# Autodesk Inventor assembly: SPE1V1 Estructura
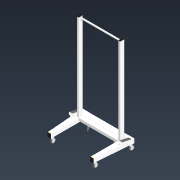
[picture p0: Inventor's stored thumbnail of the model, 180x180]
Saved by Autodesk Inventor 2021.2 (Build 252289000, 289)
## iProperties
Created: 2026-06-02
Part Number: SPE1V1 Estructura
Document SubType Name: Assembly
Designer: nelso
Mass: 32774.5 g
Surface Area: 45303.3 cm^2
Volume: 6303.93 cm^3
Density: 5.19906 g/cm^3
Author: nelso
## Documents named in this file (21)
- C:\Users\Tecnica\OneDrive\Documentos\Mecanica\Soporte-Paciente-Espinografia\Workspace\SPE1V1 Estructura.iam
- C:\Users\Tecnica\OneDrive\Documentos\Mecanica\Soporte-Paciente-Espinografia\Workspace\SP28V1 Tapacanto Delantero.ipt
- C:\Users\Tecnica\OneDrive\Documentos\Mecanica\Soporte-Paciente-Espinografia\Workspace\SP27V1 Tapacanto Superior.ipt
- C:\Users\Tecnica\OneDrive\Documentos\Mecanica\Soporte-Paciente-Espinografia\Workspace\RFPLUS8PO300.ipt
- C:\Users\Tecnica\OneDrive\Documentos\Mecanica\Soporte-Paciente-Espinografia\Workspace\SP26V1 Varilla Pedal.ipt
- C:\Users\Tecnica\OneDrive\Documentos\Mecanica\Soporte-Paciente-Espinografia\Workspace\SP23V1 Pedal Izquierdo.ipt
- C:\Users\Tecnica\OneDrive\Documentos\Mecanica\Soporte-Paciente-Espinografia\Workspace\SPE9V1 Freno.iam
- C:\Users\Tecnica\OneDrive\Documentos\Mecanica\Soporte-Paciente-Espinografia\Workspace\SP22V1 Pedal Derecho.ipt
- C:\Users\Tecnica\OneDrive\Documentos\Mecanica\Soporte-Paciente-Espinografia\Workspace\G3-100-PPP-RU.ipt
- C:\Users\Tecnica\OneDrive\Documentos\Mecanica\Soporte-Paciente-Espinografia\Workspace\DIN 555A10C.ipt
- C:\Users\Tecnica\OneDrive\Documentos\Mecanica\Soporte-Paciente-Espinografia\Workspace\DIN125-A8,4C.ipt
- C:\Users\Tecnica\OneDrive\Documentos\Mecanica\Soporte-Paciente-Espinografia\Workspace\DIN933M8X1.25L20C.ipt
- C:\Users\Tecnica\OneDrive\Documentos\Mecanica\Soporte-Paciente-Espinografia\Workspace\SP25V1 Seguro Pedales.ipt
- C:\Users\Tecnica\OneDrive\Documentos\Mecanica\Soporte-Paciente-Espinografia\Workspace\ISO7380M6X1L12I.ipt
- C:\Users\Tecnica\OneDrive\Documentos\Mecanica\Soporte-Paciente-Espinografia\Workspace\DIN137-B6.ipt
- C:\Users\Tecnica\OneDrive\Documentos\Mecanica\Soporte-Paciente-Espinografia\Workspace\ISO7380M4X0.8L12I.ipt
- C:\Users\Tecnica\OneDrive\Documentos\Mecanica\Soporte-Paciente-Espinografia\Workspace\DIN137-B4.ipt
- C:\Users\Tecnica\OneDrive\Documentos\Mecanica\Soporte-Paciente-Espinografia\Workspace\DIN555-5M4X0.8I.ipt
- C:\Users\Tecnica\OneDrive\Documentos\Mecanica\Soporte-Paciente-Espinografia\Workspace\SP24V1 Goma Pedales.ipt
- C:\Users\Tecnica\OneDrive\Documentos\Mecanica\Soporte-Paciente-Espinografia\Workspace\SPE8V1 Estructura (soldadura).iam
- C:\Users\Tecnica\OneDrive\Documentos\Mecanica\Soporte-Paciente-Espinografia\Workspace\SPE11V1 Baranda Superior (soldadura).iam
## Components (67 placed, 20 different names)
1. SPE8V1 Estructura (soldadura):1 [sub-assembly]
2. SPE9V1 Freno:1 [sub-assembly] — Flush:103, Mate:117, Mate:118, Mate:119
3. SPE9V1 Freno:2 [sub-assembly] — Flush:103, Mate:133, Mate:134
4. SP22V1 Pedal Derecho:1 — Mate:128, Mate:129, Mate:130, Mate:132, Mate:200, Mate:251, Mate:252, Mate:253, Mate:292, Mate:293, Mate:294, Mate:295, Mate:296
5. SP23V1 Pedal Izquierdo:1 — Mate:120, Mate:121, Flush:132, Mate:248, Mate:249, Mate:250, Mate:286, Mate:287, Mate:297, Mate:298, Mate:299
6. SP24V1 Goma Pedales:1 — Mate:294, Mate:295, Mate:296
7. SP24V1 Goma Pedales:2 — Mate:297, Mate:298, Mate:299
8. SP25V1 Seguro Pedales:1 — Mate:248, Mate:249, Mate:250, Mate:260, Mate:274, Mate:275, Mate:276, Mate:277
9. SP25V1 Seguro Pedales:2 — Mate:251, Mate:252, Mate:253, Mate:259, Mate:270, Mate:271, Mate:272, Mate:273
10. SP26V1 Varilla Pedal:1 — Mate:117, Mate:118, Mate:119, Mate:120, Mate:121, Mate:128, Mate:129, Mate:130, Mate:132, Mate:133, Mate:134, Mate:258, Mate:261
11. SP27V1 Tapacanto Superior:1
12. SP27V1 Tapacanto Superior:2
13. SP28V1 Tapacanto Delantero:1
14. SP28V1 Tapacanto Delantero:2
15. RFPLUS8PO300:1
16. RFPLUS8PO300:2
17. RFPLUS8PO300:3
18. RFPLUS8PO300:4
19. RFPLUS8PO300:5
20. RFPLUS8PO300:6
21. RFPLUS8PO300:17
22. RFPLUS8PO300:18
23. RFPLUS8PO300:19
24. RFPLUS8PO300:20
25. RFPLUS8PO300:21
26. RFPLUS8PO300:22
27. G3-100-PPP-RU:1
28. G3-100-PPP-RU:2
29. G3-100-PPP-RU:3
30. G3-100-PPP-RU:4
31. DIN 555A10C:1
32. DIN 555A10C:2
33. DIN 555A10C:3
34. DIN 555A10C:4
35. DIN125-A8,4C:1 — Mate:214, Mate:215
36. DIN125-A8,4C:2 — Mate:216, Mate:217
37. DIN125-A8,4C:3
38. DIN125-A8,4C:4
39. DIN933M8X1.25L20C:1 — Mate:214, Mate:215, Mate:224
40. DIN933M8X1.25L20C:2 — Mate:216, Mate:217, Mate:223
41. DIN933M8X1.25L20C:3
42. DIN933M8X1.25L20C:4
43. RFPLUS8PO300:23 — Mate:223
44. RFPLUS8PO300:24 — Mate:224
45. RFPLUS8PO300:25
46. RFPLUS8PO300:26
47. ISO7380M6X1L12I:1 — Mate:254, Mate:255, Mate:258
48. ISO7380M6X1L12I:2 — Mate:261
49. DIN137-B6:1 — Mate:254, Mate:255, Mate:259
50. DIN137-B6:2 — Mate:260
51. ISO7380M4X0.8L12I:1 — Mate:264, Mate:265, Mate:277, Mate:278, Mate:282
52. ISO7380M4X0.8L12I:2 — Mate:262, Mate:263, Mate:276, Mate:279, Mate:284
53. ISO7380M4X0.8L12I:3 — Mate:266, Mate:267, Mate:273, Mate:281, Mate:288
54. ISO7380M4X0.8L12I:4 — Mate:268, Mate:269, Mate:272, Mate:280, Mate:289
55. DIN137-B4:1 — Mate:262, Mate:263, Mate:275
56. DIN137-B4:2 — Mate:264, Mate:265, Mate:274
57. DIN137-B4:3 — Mate:268, Mate:269, Mate:270
58. DIN137-B4:4 — Mate:266, Mate:267, Mate:271
59. DIN137-B4:5 — Mate:279, Mate:285, Mate:287
60. DIN137-B4:6 — Mate:278, Mate:283, Mate:286
61. DIN137-B4:7 — Mate:280, Mate:290, Mate:293
62. DIN137-B4:8 — Mate:281, Mate:291, Mate:292
63. DIN555-5M4X0.8I:1 — Mate:282, Mate:283
64. DIN555-5M4X0.8I:2 — Mate:284, Mate:285
65. DIN555-5M4X0.8I:3 — Mate:289, Mate:290
66. DIN555-5M4X0.8I:4 — Mate:288, Mate:291
67. SPE11V1 Baranda Superior (soldadura):1 [sub-assembly]
## Relationships (167: Mate 133, Flush 33, Angle 1)
- [Mate]: SPE8V1 Estructura (soldadura):1 ↔ SP27V1 Tapacanto Superior:1
- [Flush]: SPE8V1 Estructura (soldadura):1 ↔ SP27V1 Tapacanto Superior:1
- [Mate]: SPE8V1 Estructura (soldadura):1 ↔ SP27V1 Tapacanto Superior:1
- [Flush]: SPE8V1 Estructura (soldadura):1 ↔ RFPLUS8PO300:2
- [Flush]: SPE8V1 Estructura (soldadura):1 ↔ RFPLUS8PO300:3
- [Flush]: SPE8V1 Estructura (soldadura):1 ↔ RFPLUS8PO300:4
- [Flush]: SPE8V1 Estructura (soldadura):1 ↔ RFPLUS8PO300:5
- [Flush]: SPE8V1 Estructura (soldadura):1 ↔ RFPLUS8PO300:6
- [Mate]: SPE8V1 Estructura (soldadura):1 ↔ RFPLUS8PO300:5
- [Mate]: SPE8V1 Estructura (soldadura):1 ↔ RFPLUS8PO300:6
- [Mate]: SPE8V1 Estructura (soldadura):1 ↔ RFPLUS8PO300:4
- [Mate]: SPE8V1 Estructura (soldadura):1 ↔ RFPLUS8PO300:3
- [Mate]: SPE8V1 Estructura (soldadura):1 ↔ RFPLUS8PO300:2
- [Mate]: SPE8V1 Estructura (soldadura):1 ↔ RFPLUS8PO300:1
- [Flush]: SPE8V1 Estructura (soldadura):1 ↔ RFPLUS8PO300:1
- [Mate]: SPE8V1 Estructura (soldadura):1 ↔ SPE9V1 Freno:1
- [Mate]: SPE8V1 Estructura (soldadura):1 ↔ SPE9V1 Freno:2
- Flush:103: SPE9V1 Freno:1 ↔ SPE9V1 Freno:2
- Mate:117: SPE9V1 Freno:1 ↔ SP26V1 Varilla Pedal:1
- Mate:118: SPE9V1 Freno:1 ↔ SP26V1 Varilla Pedal:1
- Mate:119: SPE9V1 Freno:1 ↔ SP26V1 Varilla Pedal:1
- Mate:120: SP23V1 Pedal Izquierdo:1 ↔ SP26V1 Varilla Pedal:1
- Mate:121: SP23V1 Pedal Izquierdo:1 ↔ SP26V1 Varilla Pedal:1
- [Mate]: SPE8V1 Estructura (soldadura):1 ↔ SPE9V1 Freno:1
- [Mate]: SPE8V1 Estructura (soldadura):1 ↔ SP26V1 Varilla Pedal:1
- [Mate] (100 mm): SPE8V1 Estructura (soldadura):1 ↔ SPE9V1 Freno:2
- [Mate] (100 mm): SPE8V1 Estructura (soldadura):1 ↔ SPE9V1 Freno:1
- Mate:128: SP22V1 Pedal Derecho:1 ↔ SP26V1 Varilla Pedal:1
- Mate:129: SP22V1 Pedal Derecho:1 ↔ SP26V1 Varilla Pedal:1
- Mate:130: SP22V1 Pedal Derecho:1 ↔ SP26V1 Varilla Pedal:1
- Mate:132: SP22V1 Pedal Derecho:1 ↔ SP26V1 Varilla Pedal:1
- Mate:133: SPE9V1 Freno:2 ↔ SP26V1 Varilla Pedal:1
- Mate:134: SPE9V1 Freno:2 ↔ SP26V1 Varilla Pedal:1
- [Flush]: SPE8V1 Estructura (soldadura):1 ↔ SP27V1 Tapacanto Superior:2
- [Mate]: SPE8V1 Estructura (soldadura):1 ↔ SP27V1 Tapacanto Superior:2
- [Mate]: SPE8V1 Estructura (soldadura):1 ↔ G3-100-PPP-RU:4
- [Mate]: SPE8V1 Estructura (soldadura):1 ↔ SP27V1 Tapacanto Superior:2
- [Mate]: SPE8V1 Estructura (soldadura):1 ↔ RFPLUS8PO300:21
- [Mate]: SPE8V1 Estructura (soldadura):1 ↔ RFPLUS8PO300:22
- [Mate]: SPE8V1 Estructura (soldadura):1 ↔ RFPLUS8PO300:20
- [Mate]: SPE8V1 Estructura (soldadura):1 ↔ RFPLUS8PO300:19
- [Mate]: SPE8V1 Estructura (soldadura):1 ↔ RFPLUS8PO300:18
- [Mate]: SPE8V1 Estructura (soldadura):1 ↔ RFPLUS8PO300:17
- [Flush]: SPE8V1 Estructura (soldadura):1 ↔ RFPLUS8PO300:17
- [Flush]: SPE8V1 Estructura (soldadura):1 ↔ RFPLUS8PO300:18
- [Flush]: SPE8V1 Estructura (soldadura):1 ↔ RFPLUS8PO300:19
- [Flush]: SPE8V1 Estructura (soldadura):1 ↔ RFPLUS8PO300:20
- [Flush]: SPE8V1 Estructura (soldadura):1 ↔ RFPLUS8PO300:21
- [Flush]: SPE8V1 Estructura (soldadura):1 ↔ RFPLUS8PO300:22
- [Mate]: SPE8V1 Estructura (soldadura):1 ↔ DIN 555A10C:3
- [Mate]: SPE8V1 Estructura (soldadura):1 ↔ DIN 555A10C:4
- [Mate]: SPE8V1 Estructura (soldadura):1 ↔ DIN 555A10C:2
- [Mate]: SPE8V1 Estructura (soldadura):1 ↔ DIN 555A10C:1
- [Mate]: SPE8V1 Estructura (soldadura):1 ↔ DIN 555A10C:1
- [Mate]: SPE8V1 Estructura (soldadura):1 ↔ DIN 555A10C:2
- [Mate]: SPE8V1 Estructura (soldadura):1 ↔ DIN 555A10C:3
- [Mate]: SPE8V1 Estructura (soldadura):1 ↔ DIN 555A10C:4
- [Flush]: SPE8V1 Estructura (soldadura):1 ↔ SP26V1 Varilla Pedal:1
- [Flush] (7.5 mm): SPE8V1 Estructura (soldadura):1
- [Flush] (7.5 mm): SPE8V1 Estructura (soldadura):1
- Flush:132: SP23V1 Pedal Izquierdo:1
- Mate:200: SP22V1 Pedal Derecho:1
- [Mate]: SPE8V1 Estructura (soldadura):1 ↔ G3-100-PPP-RU:3
- [Mate]: SPE8V1 Estructura (soldadura):1 ↔ G3-100-PPP-RU:3
- [Flush]: SPE8V1 Estructura (soldadura):1 ↔ G3-100-PPP-RU:3
- [Mate]: SPE8V1 Estructura (soldadura):1 ↔ G3-100-PPP-RU:2
- [Mate]: SPE8V1 Estructura (soldadura):1 ↔ G3-100-PPP-RU:2
- [Flush]: SPE8V1 Estructura (soldadura):1 ↔ G3-100-PPP-RU:2
- [Mate]: SPE8V1 Estructura (soldadura):1 ↔ G3-100-PPP-RU:4
- [Flush]: SPE8V1 Estructura (soldadura):1 ↔ G3-100-PPP-RU:4
- [Mate]: SPE8V1 Estructura (soldadura):1 ↔ G3-100-PPP-RU:1
- [Flush]: SPE8V1 Estructura (soldadura):1 ↔ G3-100-PPP-RU:1
- [Mate]: SPE8V1 Estructura (soldadura):1 ↔ G3-100-PPP-RU:1
- [Mate]: SPE8V1 Estructura (soldadura):1 ↔ SP28V1 Tapacanto Delantero:1
- [Flush]: SPE8V1 Estructura (soldadura):1
- [Mate]: SPE8V1 Estructura (soldadura):1
- [Flush]: SPE8V1 Estructura (soldadura):1
- [Mate] (380 mm): SPE8V1 Estructura (soldadura):1
- [Flush]: SPE8V1 Estructura (soldadura):1 ↔ SP28V1 Tapacanto Delantero:2
- [Flush]: SPE8V1 Estructura (soldadura):1 ↔ SP28V1 Tapacanto Delantero:2
- [Mate]: SPE8V1 Estructura (soldadura):1 ↔ SP28V1 Tapacanto Delantero:2
- [Flush]: SPE8V1 Estructura (soldadura):1 ↔ SP28V1 Tapacanto Delantero:1
- [Flush]: SPE8V1 Estructura (soldadura):1 ↔ SP28V1 Tapacanto Delantero:1
- Mate:214: DIN125-A8,4C:1 ↔ DIN933M8X1.25L20C:1
- Mate:215: DIN125-A8,4C:1 ↔ DIN933M8X1.25L20C:1
- Mate:216: DIN125-A8,4C:2 ↔ DIN933M8X1.25L20C:2
- Mate:217: DIN125-A8,4C:2 ↔ DIN933M8X1.25L20C:2
- [Mate]: DIN125-A8,4C:2 ↔ SPE11V1 Baranda Superior (soldadura):1
- [Mate]: DIN125-A8,4C:1 ↔ SPE11V1 Baranda Superior (soldadura):1
- [Mate]: DIN933M8X1.25L20C:1 ↔ SPE11V1 Baranda Superior (soldadura):1
- [Mate]: DIN933M8X1.25L20C:2 ↔ SPE11V1 Baranda Superior (soldadura):1
- [Mate]: SPE8V1 Estructura (soldadura):1 ↔ SPE11V1 Baranda Superior (soldadura):1
- [Flush]: SPE8V1 Estructura (soldadura):1 ↔ RFPLUS8PO300:24
- [Flush]: SPE8V1 Estructura (soldadura):1 ↔ RFPLUS8PO300:23
- Mate:223: DIN933M8X1.25L20C:2 ↔ RFPLUS8PO300:23
- Mate:224: DIN933M8X1.25L20C:1 ↔ RFPLUS8PO300:24
- [Mate]: DIN125-A8,4C:3 ↔ DIN933M8X1.25L20C:3
- [Mate]: DIN125-A8,4C:3 ↔ DIN933M8X1.25L20C:3
- [Mate]: DIN125-A8,4C:4 ↔ DIN933M8X1.25L20C:4
- [Mate]: DIN125-A8,4C:4 ↔ DIN933M8X1.25L20C:4
- [Mate]: DIN125-A8,4C:4 ↔ SPE11V1 Baranda Superior (soldadura):1
- [Mate]: DIN125-A8,4C:3 ↔ SPE11V1 Baranda Superior (soldadura):1
- [Mate]: DIN933M8X1.25L20C:3 ↔ SPE11V1 Baranda Superior (soldadura):1
- [Mate]: DIN933M8X1.25L20C:4 ↔ SPE11V1 Baranda Superior (soldadura):1
- [Mate]: DIN933M8X1.25L20C:4 ↔ RFPLUS8PO300:25
- [Mate]: DIN933M8X1.25L20C:3 ↔ RFPLUS8PO300:26
- [Mate]: SPE8V1 Estructura (soldadura):1 ↔ SPE11V1 Baranda Superior (soldadura):1
- [Flush]: SPE8V1 Estructura (soldadura):1 ↔ RFPLUS8PO300:26
- [Flush]: SPE8V1 Estructura (soldadura):1 ↔ RFPLUS8PO300:25
- [Mate]: SPE8V1 Estructura (soldadura):1 ↔ DIN933M8X1.25L20C:1
- [Mate]: SPE8V1 Estructura (soldadura):1 ↔ DIN933M8X1.25L20C:2
- [Mate]: SPE8V1 Estructura (soldadura):1 ↔ DIN933M8X1.25L20C:3
- [Mate]: SPE8V1 Estructura (soldadura):1 ↔ DIN933M8X1.25L20C:4
- [Mate]: SPE11V1 Baranda Superior (soldadura):1
- Mate:248: SP23V1 Pedal Izquierdo:1 ↔ SP25V1 Seguro Pedales:1
- Mate:249: SP23V1 Pedal Izquierdo:1 ↔ SP25V1 Seguro Pedales:1
- Mate:250: SP23V1 Pedal Izquierdo:1 ↔ SP25V1 Seguro Pedales:1
- Mate:251: SP22V1 Pedal Derecho:1 ↔ SP25V1 Seguro Pedales:2
- Mate:252: SP22V1 Pedal Derecho:1 ↔ SP25V1 Seguro Pedales:2
- Mate:253: SP22V1 Pedal Derecho:1 ↔ SP25V1 Seguro Pedales:2
- Mate:254: ISO7380M6X1L12I:1 ↔ DIN137-B6:1
- Mate:255: ISO7380M6X1L12I:1 ↔ DIN137-B6:1
- [Mate]: ISO7380M6X1L12I:2 ↔ DIN137-B6:2
- [Mate]: ISO7380M6X1L12I:2 ↔ DIN137-B6:2
- Mate:258: SP26V1 Varilla Pedal:1 ↔ ISO7380M6X1L12I:1
- Mate:259: SP25V1 Seguro Pedales:2 ↔ DIN137-B6:1
- Mate:260: SP25V1 Seguro Pedales:1 ↔ DIN137-B6:2
- Mate:261: SP26V1 Varilla Pedal:1 ↔ ISO7380M6X1L12I:2
- Mate:262: ISO7380M4X0.8L12I:2 ↔ DIN137-B4:1
- Mate:263: ISO7380M4X0.8L12I:2 ↔ DIN137-B4:1
- Mate:264: ISO7380M4X0.8L12I:1 ↔ DIN137-B4:2
- Mate:265: ISO7380M4X0.8L12I:1 ↔ DIN137-B4:2
- Mate:266: ISO7380M4X0.8L12I:3 ↔ DIN137-B4:4
- Mate:267: ISO7380M4X0.8L12I:3 ↔ DIN137-B4:4
- Mate:268: ISO7380M4X0.8L12I:4 ↔ DIN137-B4:3
- Mate:269: ISO7380M4X0.8L12I:4 ↔ DIN137-B4:3
- Mate:270: SP25V1 Seguro Pedales:2 ↔ DIN137-B4:3
- Mate:271: SP25V1 Seguro Pedales:2 ↔ DIN137-B4:4
- Mate:272: SP25V1 Seguro Pedales:2 ↔ ISO7380M4X0.8L12I:4
- Mate:273: SP25V1 Seguro Pedales:2 ↔ ISO7380M4X0.8L12I:3
- Mate:274: SP25V1 Seguro Pedales:1 ↔ DIN137-B4:2
- Mate:275: SP25V1 Seguro Pedales:1 ↔ DIN137-B4:1
- Mate:276: SP25V1 Seguro Pedales:1 ↔ ISO7380M4X0.8L12I:2
- Mate:277: SP25V1 Seguro Pedales:1 ↔ ISO7380M4X0.8L12I:1
- Mate:278: ISO7380M4X0.8L12I:1 ↔ DIN137-B4:6
- Mate:279: ISO7380M4X0.8L12I:2 ↔ DIN137-B4:5
- Mate:280: ISO7380M4X0.8L12I:4 ↔ DIN137-B4:7
- Mate:281: ISO7380M4X0.8L12I:3 ↔ DIN137-B4:8
- Mate:282: ISO7380M4X0.8L12I:1 ↔ DIN555-5M4X0.8I:1
- Mate:283: DIN137-B4:6 ↔ DIN555-5M4X0.8I:1
- Mate:284: ISO7380M4X0.8L12I:2 ↔ DIN555-5M4X0.8I:2
- Mate:285: DIN137-B4:5 ↔ DIN555-5M4X0.8I:2
- Mate:286: SP23V1 Pedal Izquierdo:1 ↔ DIN137-B4:6
- Mate:287: SP23V1 Pedal Izquierdo:1 ↔ DIN137-B4:5
- Mate:288: ISO7380M4X0.8L12I:3 ↔ DIN555-5M4X0.8I:4
- Mate:289: ISO7380M4X0.8L12I:4 ↔ DIN555-5M4X0.8I:3
- Mate:290: DIN137-B4:7 ↔ DIN555-5M4X0.8I:3
- Mate:291: DIN137-B4:8 ↔ DIN555-5M4X0.8I:4
- Mate:292: SP22V1 Pedal Derecho:1 ↔ DIN137-B4:8
- Mate:293: SP22V1 Pedal Derecho:1 ↔ DIN137-B4:7
- [Angle] (0 deg): SPE8V1 Estructura (soldadura):1 ↔ SP22V1 Pedal Derecho:1
- Mate:294: SP22V1 Pedal Derecho:1 ↔ SP24V1 Goma Pedales:1
- Mate:295: SP22V1 Pedal Derecho:1 ↔ SP24V1 Goma Pedales:1
- Mate:296: SP22V1 Pedal Derecho:1 ↔ SP24V1 Goma Pedales:1
- Mate:297: SP23V1 Pedal Izquierdo:1 ↔ SP24V1 Goma Pedales:2
- Mate:298: SP23V1 Pedal Izquierdo:1 ↔ SP24V1 Goma Pedales:2
- Mate:299: SP23V1 Pedal Izquierdo:1 ↔ SP24V1 Goma Pedales:2
## Named parameters: d314_d103 = 0 mm, d315_d104 = 0 mm, d464_d462 = 0 mm, d465_d463 = 0 mm, d466_d449 = 0 mm, d467_d450 = 0 mm, d468_d451 = 0 mm, d469_d452 = 0 mm, d470_d453 = 0 mm, d471_d454 = 0 mm, d472_d455 = 0 mm, d473_d456 = 0 mm, d500_d498 = 0 mm, d501_d499 = 0 mm
